# Autodesk Inventor assembly: Intake
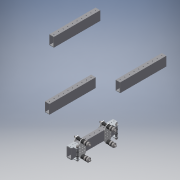
[picture p0: Inventor's stored thumbnail of the model, 180x180]
Saved by Autodesk Inventor 2018 (Build 220112000, 112)
## iProperties
Created: 2018-08-29
Part Number: Intake
Document SubType Name: Assembly
Designer: baoan
Author: baoan
## Documents named in this file (4)
- C:\Users\baoan\Documents\Inventor\Elevator\Intake.iam
- C:\Users\baoan\Documents\Inventor\Elevator\Intake_vertical.ipt
- C:\Users\baoan\Documents\Inventor\Elevator\front_bearings.iam
- C:\Users\baoan\Documents\Inventor\Elevator\Side_bearings.iam
## Components (8 placed, 3 different names)
1. Intake_vertical:1 — Mate:1
2. Intake_vertical:2 — Mate:1
3. front_bearings:1 [sub-assembly] — Mate:5, Flush:5, Flush:6
4. front_bearings:2 [sub-assembly] — Mate:3, Flush:1, Flush:2
5. Side_bearings:1 [sub-assembly] — Mate:4, Tangent:3, Tangent:4, Flush:4
6. Side_bearings:2 [sub-assembly] — Mate:2, Tangent:1, Tangent:2, Flush:3
7. Intake_vertical:3
8. Intake_vertical:4 — Mate:2, Tangent:1, Tangent:2, Mate:3, Flush:1, Flush:2, Flush:3, Mate:4, Tangent:3, Tangent:4, Flush:4, Mate:5, Flush:5, Flush:6
## Relationships (15: Flush 6, Mate 5, Tangent 4)
- Mate:1 (368.3 mm): Intake_vertical:1 ↔ Intake_vertical:2
- Mate:2: Side_bearings:2 ↔ Intake_vertical:4
- Tangent:1: Side_bearings:2 ↔ Intake_vertical:4
- Tangent:2: Side_bearings:2 ↔ Intake_vertical:4
- Mate:3: front_bearings:2 ↔ Intake_vertical:4
- Flush:1: front_bearings:2 ↔ Intake_vertical:4
- Flush:2: front_bearings:2 ↔ Intake_vertical:4
- Flush:3 (-38.1 mm): Side_bearings:2 ↔ Intake_vertical:4
- Mate:4: Side_bearings:1 ↔ Intake_vertical:4
- Tangent:3: Side_bearings:1 ↔ Intake_vertical:4
- Tangent:4: Side_bearings:1 ↔ Intake_vertical:4
- Flush:4 (38.1 mm): Side_bearings:1 ↔ Intake_vertical:4
- Mate:5: front_bearings:1 ↔ Intake_vertical:4
- Flush:5: front_bearings:1 ↔ Intake_vertical:4
- Flush:6: front_bearings:1 ↔ Intake_vertical:4
